# Autodesk Inventor assembly: final
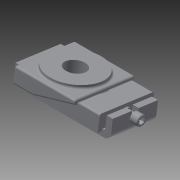
[picture p0: Inventor's stored thumbnail of the model, 180x180]
Saved by Autodesk Inventor 2015 SP2 (Build 190223200, 223)
## iProperties
Created: 2015-12-08
Part Number: final
Document SubType Name: Assembly
Designer: KC-019
Author: KC-019
## Documents named in this file (5)
- C:\Users\KC-019\Desktop\final.iam
- C:\Users\KC-019\Downloads\Base-Plate.ipt
- C:\Users\KC-019\Downloads\Sliding Block.ipt
- C:\Users\KC-019\Downloads\Adjusting Screw.ipt
- C:\Users\KC-019\Downloads\Lifting Block.ipt
## Components (4 placed, 4 different names)
1. Base-Plate:1 — Mate:1, Mate:2, Mate:3, Mate:4, Mate:5, Mate:6
2. Sliding Block:1 — Mate:1, Mate:2, Mate:7
3. Adjusting Screw:1 — Mate:3, Mate:4
4. Lifting Block:1 — Mate:5, Mate:6, Mate:7
## Relationships (7: Mate 7)
- Mate:1: Base-Plate:1 ↔ Sliding Block:1
- Mate:2: Base-Plate:1 ↔ Sliding Block:1
- Mate:3: Base-Plate:1 ↔ Adjusting Screw:1
- Mate:4: Base-Plate:1 ↔ Adjusting Screw:1
- Mate:5: Base-Plate:1 ↔ Lifting Block:1
- Mate:6: Base-Plate:1 ↔ Lifting Block:1
- Mate:7: Sliding Block:1 ↔ Lifting Block:1
